# Autodesk Inventor assembly: Mecanum_FEA
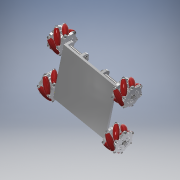
[picture p0: Inventor's stored thumbnail of the model, 180x180]
Saved by Autodesk Inventor 2018 (Build 220112000, 112)
## iProperties
Created: 2017-09-19
Part Number: Mecanum_FEA
Document SubType Name: Assembly
Designer: P136265
Author: P136265
## Documents named in this file (6)
- C:\Users\P136265\Documents\mecanum-cad\Mecanum_FEA.iam
- C:\Users\P136265\Documents\mecanum-cad\MecanumPlate_FEA.ipt
- C:\Users\P136265\Documents\Inventor\Content Center Files\R2018\en-US\DIN 625 SKF(4)\DIN 625 SKF - SKF 6004-2Z.ipt
- C:\Users\P136265\Documents\mecanum-cad\WheelShaft_FEA.ipt
- C:\Users\P136265\Documents\mecanum-cad\Mecanum_Assembly.iam
- C:\Users\P136265\Documents\Inventor\Content Center Files\R2018\en-US\ISO 4161\ISO 4161 - M20(1).ipt
## Components (26 placed, 5 different names)
1. MecanumPlate_FEA:1 — Mate:1, Mate:2, Mate:3, Mate:4, Mate:5, Mate:6, Mate:7, Mate:8, Mate:9, Mate:10, Mate:11, Mate:12, Mate:13, Mate:14, Mate:15, Mate:16, Mate:17, Mate:18, Angle:2, Mate:22, Mate:26, Mate:30, Mate:34, Mate:36, Angle:9
2. DIN 625 SKF- with two Z shields SKF 6004-2Z:1 — Mate:1, Mate:2
3. DIN 625 SKF- with two Z shields SKF 6004-2Z:2 — Mate:3, Mate:4, Angle:6, Mate:29
4. DIN 625 SKF- with two Z shields SKF 6004-2Z:3 — Mate:5, Mate:6, Angle:8, Mate:33
5. DIN 625 SKF- with two Z shields SKF 6004-2Z:4 — Mate:7, Mate:8, Mate:40
6. DIN 625 SKF- with two Z shields SKF 6004-2Z:5 — Mate:9, Mate:10, Mate:42
7. DIN 625 SKF- with two Z shields SKF 6004-2Z:6 — Mate:11, Mate:12
8. DIN 625 SKF- with two Z shields SKF 6004-2Z:7 — Mate:13, Mate:14, Mate:38
9. DIN 625 SKF- with two Z shields SKF 6004-2Z:8 — Mate:15, Mate:16, Mate:21
10. DIN 625 SKF- with two Z shields SKF 6004-2Z:9 — Mate:17, Mate:18, Angle:4, Mate:25
11. WheelShaft_FEA:1 — Angle:3, Mate:23, Mate:24, Angle:4, Mate:25, Mate:41, Mate:45
12. WheelShaft_FEA:2 — Angle:1, Mate:19, Mate:20, Angle:2, Mate:21, Mate:39, Mate:43
13. WheelShaft_FEA:3 — Angle:7, Mate:31, Mate:32, Angle:8, Mate:33, Mate:35, Mate:47
14. WheelShaft_FEA:4 — Angle:5, Mate:27, Mate:28, Angle:6, Mate:29, Mate:37, Mate:49
15. Mecanum_Assembly:1 [sub-assembly] — Angle:1, Mate:19, Mate:20, Mate:22, Mate:44
16. Mecanum_Assembly:2 [sub-assembly] — Angle:3, Mate:23, Mate:24, Mate:26, Mate:46
17. Mecanum_Assembly:3 [sub-assembly] — Angle:7, Mate:31, Mate:32, Mate:34, Mate:48
18. Mecanum_Assembly:4 [sub-assembly] — Angle:5, Mate:27, Mate:28, Mate:30, Mate:50
19. ISO 4161 M20:1 — Mate:35, Mate:36
20. ISO 4161 M20:2 — Mate:37, Mate:38
21. ISO 4161 M20:3 — Mate:39, Mate:40
22. ISO 4161 M20:4 — Mate:41, Mate:42
23. ISO 4161 M20:5 — Mate:43, Mate:44
24. ISO 4161 M20:6 — Mate:45, Mate:46
25. ISO 4161 M20:7 — Mate:47, Mate:48
26. ISO 4161 M20:8 — Mate:49, Mate:50
## Relationships (59: Mate 50, Angle 9)
- Mate:1: MecanumPlate_FEA:1 ↔ DIN 625 SKF- with two Z shields SKF 6004-2Z:1
- Mate:2: MecanumPlate_FEA:1 ↔ DIN 625 SKF- with two Z shields SKF 6004-2Z:1
- Mate:3: MecanumPlate_FEA:1 ↔ DIN 625 SKF- with two Z shields SKF 6004-2Z:2
- Mate:4: MecanumPlate_FEA:1 ↔ DIN 625 SKF- with two Z shields SKF 6004-2Z:2
- Mate:5: MecanumPlate_FEA:1 ↔ DIN 625 SKF- with two Z shields SKF 6004-2Z:3
- Mate:6: MecanumPlate_FEA:1 ↔ DIN 625 SKF- with two Z shields SKF 6004-2Z:3
- Mate:7: MecanumPlate_FEA:1 ↔ DIN 625 SKF- with two Z shields SKF 6004-2Z:4
- Mate:8: MecanumPlate_FEA:1 ↔ DIN 625 SKF- with two Z shields SKF 6004-2Z:4
- Mate:9: MecanumPlate_FEA:1 ↔ DIN 625 SKF- with two Z shields SKF 6004-2Z:5
- Mate:10: MecanumPlate_FEA:1 ↔ DIN 625 SKF- with two Z shields SKF 6004-2Z:5
- Mate:11: MecanumPlate_FEA:1 ↔ DIN 625 SKF- with two Z shields SKF 6004-2Z:6
- Mate:12: MecanumPlate_FEA:1 ↔ DIN 625 SKF- with two Z shields SKF 6004-2Z:6
- Mate:13: MecanumPlate_FEA:1 ↔ DIN 625 SKF- with two Z shields SKF 6004-2Z:7
- Mate:14: MecanumPlate_FEA:1 ↔ DIN 625 SKF- with two Z shields SKF 6004-2Z:7
- Mate:15: MecanumPlate_FEA:1 ↔ DIN 625 SKF- with two Z shields SKF 6004-2Z:8
- Mate:16: MecanumPlate_FEA:1 ↔ DIN 625 SKF- with two Z shields SKF 6004-2Z:8
- Mate:17: MecanumPlate_FEA:1 ↔ DIN 625 SKF- with two Z shields SKF 6004-2Z:9
- Mate:18: MecanumPlate_FEA:1 ↔ DIN 625 SKF- with two Z shields SKF 6004-2Z:9
- Angle:1 (0 deg): WheelShaft_FEA:2 ↔ Mecanum_Assembly:1
- Mate:19: WheelShaft_FEA:2 ↔ Mecanum_Assembly:1
- Mate:20: WheelShaft_FEA:2 ↔ Mecanum_Assembly:1
- Angle:2 (0 deg): MecanumPlate_FEA:1 ↔ WheelShaft_FEA:2
- Mate:21: DIN 625 SKF- with two Z shields SKF 6004-2Z:8 ↔ WheelShaft_FEA:2
- Mate:22 (10 mm): MecanumPlate_FEA:1 ↔ Mecanum_Assembly:1
- Angle:3 (0 deg): WheelShaft_FEA:1 ↔ Mecanum_Assembly:2
- Mate:23: WheelShaft_FEA:1 ↔ Mecanum_Assembly:2
- Mate:24: WheelShaft_FEA:1 ↔ Mecanum_Assembly:2
- Angle:4 (0 deg): DIN 625 SKF- with two Z shields SKF 6004-2Z:9 ↔ WheelShaft_FEA:1
- Mate:25: DIN 625 SKF- with two Z shields SKF 6004-2Z:9 ↔ WheelShaft_FEA:1
- Mate:26 (10 mm): MecanumPlate_FEA:1 ↔ Mecanum_Assembly:2
- Angle:5 (0 deg): WheelShaft_FEA:4 ↔ Mecanum_Assembly:4
- Mate:27: WheelShaft_FEA:4 ↔ Mecanum_Assembly:4
- Mate:28: WheelShaft_FEA:4 ↔ Mecanum_Assembly:4
- Angle:6 (0 deg): DIN 625 SKF- with two Z shields SKF 6004-2Z:2 ↔ WheelShaft_FEA:4
- Mate:29: DIN 625 SKF- with two Z shields SKF 6004-2Z:2 ↔ WheelShaft_FEA:4
- Mate:30 (10 mm): MecanumPlate_FEA:1 ↔ Mecanum_Assembly:4
- Angle:7 (0 deg): WheelShaft_FEA:3 ↔ Mecanum_Assembly:3
- Mate:31: WheelShaft_FEA:3 ↔ Mecanum_Assembly:3
- Mate:32: WheelShaft_FEA:3 ↔ Mecanum_Assembly:3
- Angle:8 (0 deg): DIN 625 SKF- with two Z shields SKF 6004-2Z:3 ↔ WheelShaft_FEA:3
- Mate:33: DIN 625 SKF- with two Z shields SKF 6004-2Z:3 ↔ WheelShaft_FEA:3
- Mate:34 (10 mm): MecanumPlate_FEA:1 ↔ Mecanum_Assembly:3
- Mate:35: WheelShaft_FEA:3 ↔ ISO 4161 M20:1
- Mate:36: MecanumPlate_FEA:1 ↔ ISO 4161 M20:1
- Mate:37: WheelShaft_FEA:4 ↔ ISO 4161 M20:2
- Mate:38: DIN 625 SKF- with two Z shields SKF 6004-2Z:7 ↔ ISO 4161 M20:2
- Mate:39: WheelShaft_FEA:2 ↔ ISO 4161 M20:3
- Mate:40: DIN 625 SKF- with two Z shields SKF 6004-2Z:4 ↔ ISO 4161 M20:3
- Mate:41: WheelShaft_FEA:1 ↔ ISO 4161 M20:4
- Mate:42: DIN 625 SKF- with two Z shields SKF 6004-2Z:5 ↔ ISO 4161 M20:4
- Mate:43: WheelShaft_FEA:2 ↔ ISO 4161 M20:5
- Mate:44: Mecanum_Assembly:1 ↔ ISO 4161 M20:5
- Mate:45: WheelShaft_FEA:1 ↔ ISO 4161 M20:6
- Mate:46: Mecanum_Assembly:2 ↔ ISO 4161 M20:6
- Mate:47: WheelShaft_FEA:3 ↔ ISO 4161 M20:7
- Mate:48: Mecanum_Assembly:3 ↔ ISO 4161 M20:7
- Mate:49: WheelShaft_FEA:4 ↔ ISO 4161 M20:8
- Mate:50: Mecanum_Assembly:4 ↔ ISO 4161 M20:8
- Angle:9 (0 deg): MecanumPlate_FEA:1
